# Autodesk Inventor assembly: V3Climb
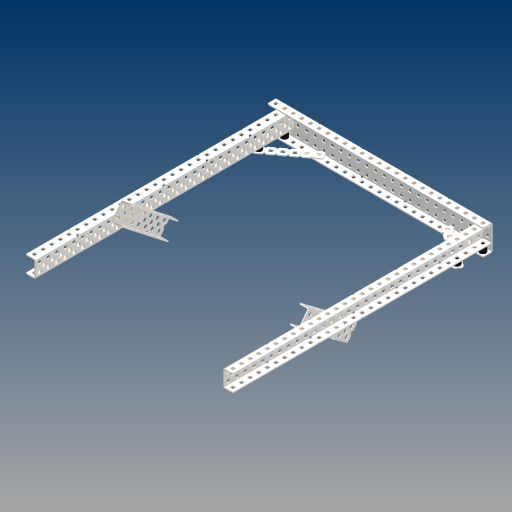
[picture p0: Inventor's stored thumbnail of the model, 512x512]
Saved by Autodesk Inventor 2023 (Build 270158000, 158)
## iProperties
Created: 2023-10-21
Part Number: V3Climb
Document SubType Name: Assembly
Designer: eddie
Author: eddie
## Documents named in this file (8)
- C:\Users\eddie\Documents\81208X-Over-Under-CAD\V3\V3Climb.iam
- C:\Users\eddie\Documents\81208X-Over-Under-CAD\VEX-CAD-Inventor-1.4.0\Structure\C Channel\Aluminum 1x2x1\Alu C 1x2x1x30.ipt
- C:\Users\eddie\Documents\81208X-Over-Under-CAD\VEX-CAD-Inventor-1.4.0\Structure\C Channel\Aluminum 1x3x1\Alu C 1x3x1x25.ipt
- C:\Users\eddie\Documents\81208X-Over-Under-CAD\VEX-CAD-Inventor-1.4.0\Motion\Spacers\Spacer Nylon .375 OD\NSpacer .375 OD x .375.ipt
- C:\Users\eddie\Documents\81208X-Over-Under-CAD\VEX-CAD-Inventor-1.4.0\Motion\Spacers\Spacer Nylon .375 OD.ipt
- C:\Users\eddie\Documents\81208X-Over-Under-CAD\VEX-CAD-Inventor-1.4.0\Motion\Spacers\Spacer Nylon .375 OD\NSpacer .375 OD x .250.ipt
- C:\Users\eddie\Documents\81208X-Over-Under-CAD\VEX-CAD-Inventor-1.4.0\Structure\Plate\Aluminum\Alu Plate 1x6.ipt
- C:\Users\eddie\Documents\81208X-Over-Under-CAD\VEX-CAD-Inventor-1.4.0\Structure\C Channel\Aluminum 1x2x1\Alu C 1x2x1x7.ipt
## Components (11 placed, 6 different names)
1. Alu C 1x2x1x30:2 — Insert:1, Insert:6, Insert:12
2. Alu C 1x3x1x25:1 — Insert:1, Insert:3, Insert:7, Insert:8
3. NSpacer .375 OD x .375:1 — Insert:3
4. NSpacer .375 OD x .250:4 — Insert:6, Insert:11
5. Alu C 1x2x1x30:3 — Insert:7, Insert:9, Insert:13
6. NSpacer .375 OD x .250:5 — Insert:9, Insert:10
7. NSpacer .375 OD x .375:6 — Insert:8
8. Alu Plate 1x6:1 — Insert:10
9. Alu Plate 1x6:2 — Insert:11
10. Alu C 1x2x1x7:1 — Insert:12
11. Alu C 1x2x1x7:2 — Insert:13
## Relationships (10: Insert 10)
- Insert:1: Alu C 1x2x1x30:2 ↔ Alu C 1x3x1x25:1
- Insert:3: Alu C 1x3x1x25:1 ↔ NSpacer .375 OD x .375:1
- Insert:6: Alu C 1x2x1x30:2 ↔ NSpacer .375 OD x .250:4
- Insert:7: Alu C 1x3x1x25:1 ↔ Alu C 1x2x1x30:3
- Insert:8: Alu C 1x3x1x25:1 ↔ NSpacer .375 OD x .375:6
- Insert:9: Alu C 1x2x1x30:3 ↔ NSpacer .375 OD x .250:5
- Insert:10: NSpacer .375 OD x .250:5 ↔ Alu Plate 1x6:1
- Insert:11: NSpacer .375 OD x .250:4 ↔ Alu Plate 1x6:2
- Insert:12: Alu C 1x2x1x30:2 ↔ Alu C 1x2x1x7:1
- Insert:13: Alu C 1x2x1x30:3 ↔ Alu C 1x2x1x7:2
